# Autodesk Inventor assembly: Z-head-assembly-IKO-T1
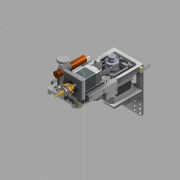
[picture p0: Inventor's stored thumbnail of the model, 180x180]
Saved by Autodesk Inventor 2016 (Build 200138000, 138)
## iProperties
Created: 2015-05-08
Part Number: Z-head-assembly-IKO-T1
Document SubType Name: Assembly
Designer: ax
Mass: 531.775 g
Surface Area: 986.994 cm^2
Volume: 148.74 cm^3
Density: 3.5752 g/cm^3
Author: ax
## Documents named in this file (36)
- C:\Users\as\Documents\Inventor\mintplacer-export\Z-head-assembly-IKO-T1.iam
- C:\Users\as\Documents\Inventor\mintplacer-export\Z-head-baseplate-IKO.ipt
- C:\Users\as\Documents\Inventor\mintplacer-export\BSPG15_60__40_.iam
- C:\Users\as\Documents\Inventor\mintplacer-export\C-head-base.ipt
- C:\Users\as\Documents\Inventor\mintplacer-export\C-head-side.ipt
- C:\Users\as\Documents\Inventor\mintplacer-export\GT2_20tooth.ipt
- C:\Users\as\Documents\Inventor\mintplacer-export\GT2-belt-2MR-200-06.ipt
- C:\Users\as\Documents\Inventor\mintplacer-export\HTD-5M-belt-clamp.ipt
- C:\Users\as\Documents\Inventor\mintplacer-export\GT2 belt clamp.ipt
- C:\Users\as\Documents\Inventor\mintplacer-export\nozzle-assembly.iam
- C:\Users\as\Documents\Inventor\mintplacer-export\Nanotec-ST4118S1404.iam
- C:\Users\as\Documents\Inventor\mintplacer-export\c-head-flange.ipt
- C:\Users\as\Documents\Inventor\mintplacer-export\Z-head-assembly-IKO-T1\Design Accelerator\Bolted Connection3.iam
- C:\Users\as\Documents\Inventor\mintplacer-export\Z-head-assembly-IKO-T1\Design Accelerator\Bolted Connection4.iam
- C:\Users\as\Documents\Inventor\mintplacer-export\Z-head-assembly-IKO-T1\Design Accelerator\Bolted Connection5.iam
- C:\Users\as\Documents\Inventor\mintplacer-export\Z-head-assembly-IKO-T1\Design Accelerator\Bolted Connection6.iam
- C:\Users\as\Documents\Inventor\mintplacer-export\Z-head-assembly-IKO-T1\Design Accelerator\Bolted Connection7.iam
- C:\Users\as\Documents\Inventor\mintplacer-export\small-tact-switch.ipt
- C:\Users\as\Documents\Inventor\mintplacer-export\Z-head-assembly-IKO-T1\Design Accelerator\Bolted Connection8.iam
- C:\Users\as\Documents\Inventor\Content Center Files\R2016\en-US\ISO 4762(1)\DIN EN ISO 4762 - M3 x 12.ipt
- C:\Users\as\Documents\Inventor\mintplacer-export\cam-flying.iam
- C:\Users\as\Documents\Inventor\mintplacer-export\Z-head-assembly-IKO-T1\Design Accelerator\Bolted Connection13.iam
- C:\Users\as\Documents\Inventor\mintplacer-export\Z-head-assembly-IKO-T1\Design Accelerator\Bolted Connection14.iam
- C:\Users\as\Documents\Inventor\mintplacer-export\Z-head-sideplate.ipt
- C:\Users\as\Documents\Inventor\mintplacer-export\Z-head-topplate.ipt
- C:\Users\as\Documents\Inventor\mintplacer-export\Z-head-beltmount.ipt
- C:\Users\as\Documents\Inventor\mintplacer-export\Z-head-assembly-IKO-T1\Design Accelerator\Bolted Connection15.iam
- C:\Users\as\Documents\Inventor\mintplacer-export\Z-head-assembly-IKO-T1\Design Accelerator\Bolted Connection16.iam
- C:\Users\as\Documents\Inventor\mintplacer-export\Z-head-assembly-IKO-T1\Design Accelerator\Bolted Connection17.iam
- C:\Users\as\Documents\Inventor\mintplacer-export\Z-head-assembly-IKO-T1\Design Accelerator\Bolted Connection18.iam
- C:\Users\as\Documents\Inventor\mintplacer-export\Nanotec-NEMA8-st2018s0604\st2018s0604.iam
- C:\Users\as\Documents\Inventor\mintplacer-export\Z-linear-encoder.ipt
- C:\Users\as\Documents\Inventor\mintplacer-export\Z-encoder-mounting-plate.ipt
- C:\Users\as\Documents\Inventor\mintplacer-export\z-linear-encoder-strip-standoff.ipt
- C:\Users\as\Documents\Inventor\mintplacer-export\encoder-linear-strip.ipt
- C:\Users\as\Documents\Inventor\mintplacer-export\Z-head-assembly-IKO-T1\Design Accelerator\Bolted Connection19.iam
## Components (48 placed, 23 different names)
1. Z-head-baseplate-IKO:1 — Mate:1, Flush:1, Flush:7, Mate:5, Mate:10, Mate:70, Mate:71, Mate:74, Mate:76, Mate:110, Flush:31, Mate:111, Mate:112, Mate:116, Angle:1, Mate:118, Flush:36, Flush:37, Flush:38, Mate:121, Mate:133, Mate:135, Flush:43, Flush:44, Mate:152, Flush:45, Flush:46, Flush:47, Mate:153, Flush:48, Mate:155, Mate:156
2. HTD-5M-belt-clamp:1 — Mate:131, Flush:42
3. Nanotec-ST4118S1404:2 [sub-assembly] — Mate:5, Mate:10, Cylindrical:1, Mate:72, Mate:73, Mate:75, Flush:33, Mate:117
4. GT2_20tooth:1 — Mate:4, Cylindrical:1
5. BSPG15_60__40_:1 [sub-assembly] — Mate:1, Flush:1, Flush:3, Mate:11, Flush:19, Flush:20, Mate:84, Mate:86, Mate:122, Flush:44
6. c-head-flange:1 — Flush:14, Flush:15, Mate:11, Mate:12, Flush:17, Flush:19, Mate:32, Flush:20, Mate:83, Mate:85, Mate:87, Mate:88, Mate:130, Mate:145
7. C-head-base:1 — Flush:3, Flush:13, Flush:14, Flush:15, Flush:18, Mate:17, Mate:78, Mate:142, Mate:143, Angle:2
8. C-head-side:1 — Mate:7, Flush:11, Flush:13, Mate:12, Flush:17, Flush:18, Mate:17, Mate:77, Flush:34, Mate:129
9. st2018s0604:1 [sub-assembly] — Mate:142, Mate:143, Mate:144, Angle:2
10. nozzle-assembly:1 [sub-assembly] — Mate:144
11. GT2 belt clamp:1 — Mate:7, Flush:11, Flush:34, Mate:127, Mate:128
12. Bolted Connection:3 [sub-assembly] — Mate:77, Mate:78
13. Bolted Connection:4 [sub-assembly] — Mate:129, Mate:130
14. Bolted Connection:5 [sub-assembly] — Mate:127, Mate:128
15. Bolted Connection:6 [sub-assembly] — Mate:83, Mate:84
16. Bolted Connection:7 [sub-assembly] — Mate:85, Mate:86
17. small-tact-switch:1 — Mate:32, Mate:145
18. Bolted Connection:8 [sub-assembly] — Mate:87, Mate:88
19. small-tact-switch:2
20. small-tact-switch:3
21. DIN EN ISO 4762 M3 x 12:1 — Mate:70, Mate:117
22. DIN EN ISO 4762 M3 x 12:2 — Mate:71, Mate:72
23. DIN EN ISO 4762 M3 x 12:3 — Mate:74, Mate:75
24. DIN EN ISO 4762 M3 x 12:4 — Mate:73, Mate:76
25. cam-flying:1 [sub-assembly] — Mate:110, Flush:31, Mate:111, Mate:113
26. Bolted Connection:13 [sub-assembly] — Mate:112, Mate:113
27. Bolted Connection:14 [sub-assembly] — Mate:121, Mate:122
28. Z-head-sideplate:1 — Mate:119, Flush:39, Flush:40, Mate:120, Mate:134, Mate:138
29. Z-head-topplate:1 — Flush:36, Flush:37, Flush:38, Mate:119, Flush:39, Flush:40, Flush:41, Mate:132, Mate:140
30. Z-head-beltmount:1 — Flush:41, Mate:120, Mate:131, Flush:42, Flush:43, Mate:139, Mate:141
31. Bolted Connection:15 [sub-assembly] — Mate:132, Mate:133
32. Bolted Connection:16 [sub-assembly] — Mate:134, Mate:135
33. Bolted Connection:17 [sub-assembly] — Mate:140, Mate:141
34. Bolted Connection:18 [sub-assembly] — Mate:138, Mate:139
35. Z-linear-encoder:1 — Mate:155, Mate:156, Flush:49, Mate:157, Mate:158
36. Z-encoder-mounting-plate:1 — Flush:49
37. z-linear-encoder-strip-standoff:1 — Mate:152, Flush:45, Flush:46
38. z-linear-encoder-strip-standoff:2 — Flush:47, Mate:153, Mate:154
39. encoder-linear-strip:1 — Mate:154, Flush:48
40. Bolted Connection:19 [sub-assembly] — Mate:157, Mate:158
41. GT2-belt-2MR-200-06:1 — Mate:4, Mate:118
42. GT2-belt-2MR-200-06:2
43. GT2-belt-2MR-200-06:3
44. GT2-belt-2MR-200-06:4
45. GT2-belt-2MR-200-06:5
46. GT2-belt-2MR-200-06:6
47. GT2-belt-2MR-200-06:7
48. GT2-belt-2MR-200-06:8
## Component patterns: (8 elements, first: GT2-belt-2MR-200-06:1)
## Relationships (92: Mate 59, Flush 30, Angle 2, CylindricalJoint 1)
- Mate:1: Z-head-baseplate-IKO:1 ↔ BSPG15_60__40_:1
- Flush:1: Z-head-baseplate-IKO:1 ↔ BSPG15_60__40_:1
- Flush:3: BSPG15_60__40_:1 ↔ C-head-base:1
- Mate:4 (1 mm): GT2_20tooth:1 ↔ GT2-belt-2MR-200-06:1
- Flush:7 (-6.3662 mm): Z-head-baseplate-IKO:1
- Mate:5 (-21 mm): Z-head-baseplate-IKO:1 ↔ Nanotec-ST4118S1404:2
- Flush:8 (-1.15 mm)
- Mate:7: C-head-side:1 ↔ GT2 belt clamp:1
- Flush:11: C-head-side:1 ↔ GT2 belt clamp:1
- Flush:13: C-head-base:1 ↔ C-head-side:1
- Mate:10: Z-head-baseplate-IKO:1 ↔ Nanotec-ST4118S1404:2
- Cylindrical:1: Nanotec-ST4118S1404:2 ↔ GT2_20tooth:1
- Flush:14: c-head-flange:1 ↔ C-head-base:1
- Flush:15: c-head-flange:1 ↔ C-head-base:1
- Mate:11: BSPG15_60__40_:1 ↔ c-head-flange:1
- Mate:12: c-head-flange:1 ↔ C-head-side:1
- Flush:17: c-head-flange:1 ↔ C-head-side:1
- Flush:18: C-head-base:1 ↔ C-head-side:1
- Flush:19: BSPG15_60__40_:1 ↔ c-head-flange:1
- Mate:17: C-head-base:1 ↔ C-head-side:1
- Mate:32: c-head-flange:1 ↔ small-tact-switch:1
- Flush:20: BSPG15_60__40_:1 ↔ c-head-flange:1
- Mate:70: Z-head-baseplate-IKO:1 ↔ DIN EN ISO 4762 M3 x 12:1
- Mate:71: Z-head-baseplate-IKO:1 ↔ DIN EN ISO 4762 M3 x 12:2
- Mate:72: Nanotec-ST4118S1404:2 ↔ DIN EN ISO 4762 M3 x 12:2
- Mate:73: Nanotec-ST4118S1404:2 ↔ DIN EN ISO 4762 M3 x 12:4
- Mate:74: Z-head-baseplate-IKO:1 ↔ DIN EN ISO 4762 M3 x 12:3
- Mate:75: Nanotec-ST4118S1404:2 ↔ DIN EN ISO 4762 M3 x 12:3
- Mate:76: Z-head-baseplate-IKO:1 ↔ DIN EN ISO 4762 M3 x 12:4
- Mate:77: C-head-side:1 ↔ Bolted Connection:3
- Mate:78: C-head-base:1 ↔ Bolted Connection:3
- Mate:83: c-head-flange:1 ↔ Bolted Connection:6
- Mate:84: BSPG15_60__40_:1 ↔ Bolted Connection:6
- Mate:85: c-head-flange:1 ↔ Bolted Connection:7
- Mate:86: BSPG15_60__40_:1 ↔ Bolted Connection:7
- Mate:87: c-head-flange:1 ↔ Bolted Connection:8
- Mate:88: c-head-flange:1 ↔ Bolted Connection:8
- Mate:110: Z-head-baseplate-IKO:1 ↔ cam-flying:1
- Flush:31: Z-head-baseplate-IKO:1 ↔ cam-flying:1
- Mate:111: Z-head-baseplate-IKO:1 ↔ cam-flying:1
- Mate:112: Z-head-baseplate-IKO:1 ↔ Bolted Connection:13
- Mate:113: cam-flying:1 ↔ Bolted Connection:13
- Mate:116: Z-head-baseplate-IKO:1
- Angle:1 (0 deg): Z-head-baseplate-IKO:1
- Flush:32 (-79 mm)
- Flush:33 (-21 mm): Nanotec-ST4118S1404:2
- Mate:117: Nanotec-ST4118S1404:2 ↔ DIN EN ISO 4762 M3 x 12:1
- Flush:34: C-head-side:1 ↔ GT2 belt clamp:1
- Mate:118 (-7 mm): Z-head-baseplate-IKO:1 ↔ GT2-belt-2MR-200-06:1
- Flush:36: Z-head-baseplate-IKO:1 ↔ Z-head-topplate:1
- Flush:37: Z-head-baseplate-IKO:1 ↔ Z-head-topplate:1
- Flush:38: Z-head-baseplate-IKO:1 ↔ Z-head-topplate:1
- Mate:119: Z-head-sideplate:1 ↔ Z-head-topplate:1
- Flush:39: Z-head-sideplate:1 ↔ Z-head-topplate:1
- Flush:40: Z-head-sideplate:1 ↔ Z-head-topplate:1
- Flush:41: Z-head-topplate:1 ↔ Z-head-beltmount:1
- Mate:120: Z-head-sideplate:1 ↔ Z-head-beltmount:1
- Mate:121: Z-head-baseplate-IKO:1 ↔ Bolted Connection:14
- Mate:122: BSPG15_60__40_:1 ↔ Bolted Connection:14
- Mate:127: GT2 belt clamp:1 ↔ Bolted Connection:5
- Mate:128: GT2 belt clamp:1 ↔ Bolted Connection:5
- Mate:129: C-head-side:1 ↔ Bolted Connection:4
- Mate:130: c-head-flange:1 ↔ Bolted Connection:4
- Mate:131: HTD-5M-belt-clamp:1 ↔ Z-head-beltmount:1
- Flush:42: HTD-5M-belt-clamp:1 ↔ Z-head-beltmount:1
- Mate:132: Z-head-topplate:1 ↔ Bolted Connection:15
- Mate:133: Z-head-baseplate-IKO:1 ↔ Bolted Connection:15
- Mate:134: Z-head-sideplate:1 ↔ Bolted Connection:16
- Mate:135: Z-head-baseplate-IKO:1 ↔ Bolted Connection:16
- Flush:43 (-35 mm): Z-head-baseplate-IKO:1 ↔ Z-head-beltmount:1
- Mate:138: Z-head-sideplate:1 ↔ Bolted Connection:18
- Mate:139: Z-head-beltmount:1 ↔ Bolted Connection:18
- Mate:140: Z-head-topplate:1 ↔ Bolted Connection:17
- Mate:141: Z-head-beltmount:1 ↔ Bolted Connection:17
- Mate:142: C-head-base:1 ↔ st2018s0604:1
- Mate:143: C-head-base:1 ↔ st2018s0604:1
- Mate:144: st2018s0604:1 ↔ nozzle-assembly:1
- Flush:44 (2 mm): Z-head-baseplate-IKO:1 ↔ BSPG15_60__40_:1
- Mate:145: c-head-flange:1 ↔ small-tact-switch:1
- Mate:152: Z-head-baseplate-IKO:1 ↔ z-linear-encoder-strip-standoff:1
- Flush:45 (4 mm): Z-head-baseplate-IKO:1 ↔ z-linear-encoder-strip-standoff:1
- Flush:46 (-47.5 mm): Z-head-baseplate-IKO:1 ↔ z-linear-encoder-strip-standoff:1
- Flush:47 (4 mm): Z-head-baseplate-IKO:1 ↔ z-linear-encoder-strip-standoff:2
- Mate:153: Z-head-baseplate-IKO:1 ↔ z-linear-encoder-strip-standoff:2
- Mate:154: z-linear-encoder-strip-standoff:2 ↔ encoder-linear-strip:1
- Flush:48 (4 mm): Z-head-baseplate-IKO:1 ↔ encoder-linear-strip:1
- Mate:155 (2 mm): Z-head-baseplate-IKO:1 ↔ Z-linear-encoder:1
- Mate:156 (-13.5 mm): Z-head-baseplate-IKO:1 ↔ Z-linear-encoder:1
- Flush:49 (1 mm): Z-linear-encoder:1 ↔ Z-encoder-mounting-plate:1
- Mate:157: Z-linear-encoder:1 ↔ Bolted Connection:19
- Mate:158: Z-linear-encoder:1 ↔ Bolted Connection:19
- Angle:2 (0 deg): C-head-base:1 ↔ st2018s0604:1
## Named parameters: pulleyTeeth = 20, cPulley = 40 mm, dPulley = 12.7324 mm, beltThickness = 1.15 mm
